# Autodesk Inventor assembly: door1_cover
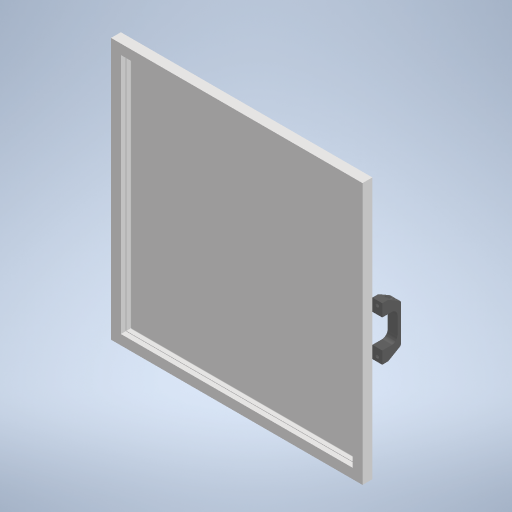
[picture p0: Inventor's stored thumbnail of the model, 512x512]
Saved by Autodesk Inventor 2023.5 (Build 275446000, 446)
## iProperties
Created: 2025-04-17
Part Number: door1_cover
Document SubType Name: Assembly
Designer: LENOVO
Author: LENOVO
## Documents named in this file (4)
- E:\filedata\invertorfile\tudien\door1_cover.iam
- E:\filedata\invertorfile\tudien\door1.ipt
- E:\filedata\invertorfile\tudien\coverdoor1.ipt
- E:\filedata\invertorfile\tudien\Handle 108 mm\Handle 108 mm.ipt
## Components (3 placed, 3 different names)
1. door1:1 — Mate:1, Flush:1, Mate:2, Mate:3, Mate:4, Flush:2
2. coverdoor1:1 — Mate:1, Flush:1, Mate:2
3. Handle 108 mm:1 — Mate:3, Mate:4, Flush:2
## Relationships (6: Mate 4, Flush 2)
- Mate:1: door1:1 ↔ coverdoor1:1
- Flush:1: door1:1 ↔ coverdoor1:1
- Mate:2: door1:1 ↔ coverdoor1:1
- Mate:3: door1:1 ↔ Handle 108 mm:1
- Mate:4: door1:1 ↔ Handle 108 mm:1
- Flush:2 (211 mm): door1:1 ↔ Handle 108 mm:1
